# Autodesk Inventor assembly: Carriage Streamlined
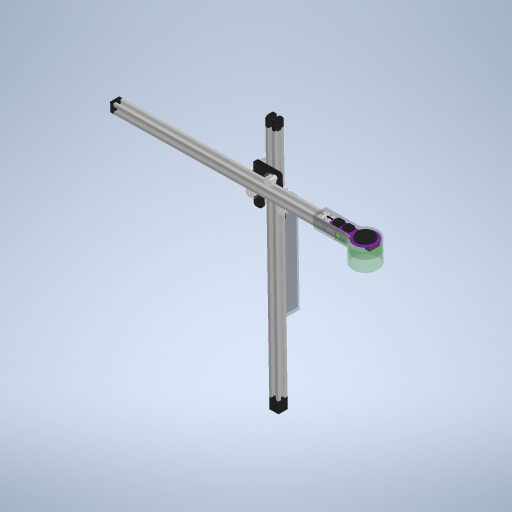
[picture p0: Inventor's stored thumbnail of the model, 512x512]
Saved by Autodesk Inventor 2024 (Build 280153000, 153)
## iProperties
Created: 2022-12-12
Part Number: Carriage Streamlined
Document SubType Name: Assembly
Designer: AdminForWorker
Title: Carriage Streamlined v19
Author: AdminForWorker
## Documents named in this file (23)
- C:\Users\lunima\Desktop\DOSYN\3D Model\Dosyn.iam
- C:\Users\lunima\Desktop\DOSYN\3D Model\Carriage\Routed Spacer.ipt
- C:\Users\lunima\Desktop\DOSYN\3D Model\Carriage\Wheel.iam
- C:\Users\lunima\Desktop\DOSYN\3D Model\Carriage\Wheel_1.iam
- C:\Users\lunima\Desktop\DOSYN\3D Model\Carriage\Wheel_2.iam
- C:\Users\lunima\Desktop\DOSYN\3D Model\Carriage\Wheel_3.iam
- C:\Users\lunima\Desktop\DOSYN\3D Model\Carriage\Wheel_4.iam
- C:\Users\lunima\Desktop\DOSYN\3D Model\Carriage\Wheel_5.iam
- C:\Users\lunima\Desktop\DOSYN\3D Model\Carriage\Carriage.ipt
- C:\Users\lunima\Desktop\DOSYN\3D Model\Carriage\Component8.ipt
- C:\Users\lunima\Desktop\DOSYN\3D Model\Carriage\Belt Clip.ipt
- C:\Users\lunima\Desktop\DOSYN\3D Model\Carriage\Pogo Pin Clip.ipt
- C:\Users\lunima\Desktop\DOSYN\3D Model\Main Structure\2020Z.ipt
- C:\Users\lunima\Desktop\DOSYN\3D Model\Main Structure\Side Lid.ipt
- C:\Users\lunima\Desktop\DOSYN\3D Model\Main Structure\Base.ipt
- C:\Users\lunima\Desktop\DOSYN\3D Model\Main Structure\Pulley Mount.ipt
- C:\Users\lunima\Desktop\DOSYN\3D Model\Counterweight\Counterweight Belt Clip.ipt
- C:\Users\lunima\Desktop\DOSYN\3D Model\Counterweight\Counterweight Enclosure.ipt
- C:\Users\lunima\Desktop\DOSYN\3D Model\Counterweight\Counterweight Flex Tab.ipt
- C:\Users\lunima\Desktop\DOSYN\3D Model\Counterweight\Counterweight Lid.ipt
- C:\Users\lunima\Desktop\DOSYN\3D Model\LED Cover\Dosyn LED.iam
- C:\Users\lunima\Desktop\DOSYN\3D Model\Main Structure\Hot Pipe.ipt
- C:\Users\lunima\Desktop\DOSYN\3D Model\Carriage\Pogo Pin.ipt
## Components (29 placed, 17 different names)
1. Routed Spacer:1 — 旋转:9, 旋转:10
2. Routed Spacer:2 — 旋转:12, 旋转:13
3. Wheel:1 [sub-assembly] — 旋转:13
4. Wheel:2 [sub-assembly] — 旋转:14
5. Wheel:3 [sub-assembly] — 旋转:10
6. Routed Spacer:4 — 旋转:7, 旋转:8
7. Routed Spacer:5 — 旋转:5, 旋转:6
8. Routed Spacer:6 — 刚性:1, 旋转:4
9. Wheel:4 [sub-assembly] — 旋转:8
10. Wheel:5 [sub-assembly] — 旋转:4
11. Wheel:6 [sub-assembly] — 旋转:6
12. Carriage:1 — 旋转:1, 旋转:2, 旋转:3, 刚性:1, 旋转:5, 旋转:7, 旋转:9, 旋转:11, 旋转:12, 配合:1, 配合:2, 表面齐平:1, 配合:3, 表面齐平:2
13. Component8:1 — 旋转:11, 旋转:14
14. Belt Clip:1 — 旋转:1, 配合:1
15. Pogo Pin Clip:1 — 旋转:2
16. Pogo Pin Clip:2 — 旋转:3, 配合:15, 配合:16, 配合:17, 配合:18, 配合:19, 配合:20
17. 2020Z:1 — 配合:3, 表面齐平:2, 旋转:16, 表面齐平:4, 旋转:17, 表面齐平:5, 配合:10, 表面齐平:6
18. 2020Z:2 — 配合:2, 表面齐平:1, 旋转:15, 表面齐平:3, 配合:11, 配合:12, 配合:13, 配合:14, 表面齐平:7
19. Side Lid:1 — 旋转:15, 表面齐平:3
20. Base:1 — 旋转:16, 表面齐平:4
21. Pulley Mount:1 — 旋转:17, 表面齐平:5
22. Counterweight Belt Clip:1 — 旋转:18, 配合:7
23. Counterweight Enclosure:1 — 配合:4, 配合:5, 配合:6, 旋转:18, 配合:7, 配合:8, 配合:9, 配合:10, 表面齐平:6
24. Counterweight Flex Tab:1 — 配合:4, 配合:5, 配合:6
25. Counterweight Lid:1 — 配合:8, 配合:9
26. Dosyn LED:1 [sub-assembly] — 配合:11, 配合:12, 配合:13
27. Hot Pipe:1 — 配合:14, 表面齐平:7
28. Pogo Pin:1 — 配合:15, 配合:16, 配合:17
29. Pogo Pin:2 — 配合:18, 配合:19, 配合:20
## Relationships (46: Mate 20, RevoluteJoint 18, Flush 7, WeldJoint 1)
- 旋转:1 [RevoluteJoint]: Carriage:1 ↔ Belt Clip:1
- 旋转:2 [RevoluteJoint]: Carriage:1 ↔ Pogo Pin Clip:1
- 旋转:3 [RevoluteJoint]: Carriage:1 ↔ Pogo Pin Clip:2
- 刚性:1 [WeldJoint]: Routed Spacer:6 ↔ Carriage:1
- 旋转:4 [RevoluteJoint]: Routed Spacer:6 ↔ Wheel:5
- 旋转:5 [RevoluteJoint]: Routed Spacer:5 ↔ Carriage:1
- 旋转:6 [RevoluteJoint]: Routed Spacer:5 ↔ Wheel:6
- 旋转:7 [RevoluteJoint]: Routed Spacer:4 ↔ Carriage:1
- 旋转:8 [RevoluteJoint]: Routed Spacer:4 ↔ Wheel:4
- 旋转:9 [RevoluteJoint]: Routed Spacer:1 ↔ Carriage:1
- 旋转:10 [RevoluteJoint]: Routed Spacer:1 ↔ Wheel:3
- 旋转:11 [RevoluteJoint]: Carriage:1 ↔ Component8:1
- 旋转:12 [RevoluteJoint]: Routed Spacer:2 ↔ Carriage:1
- 旋转:13 [RevoluteJoint]: Routed Spacer:2 ↔ Wheel:1
- 旋转:14 [RevoluteJoint]: Wheel:2 ↔ Component8:1
- 配合:1 [Mate]: Carriage:1 ↔ Belt Clip:1
- 配合:2 [Mate] (1.5 mm): Carriage:1 ↔ 2020Z:2
- 表面齐平:1 [Flush] (18.85 mm): Carriage:1 ↔ 2020Z:2
- 配合:3 [Mate] (1.5 mm): Carriage:1 ↔ 2020Z:1
- 表面齐平:2 [Flush] (18.85 mm): Carriage:1 ↔ 2020Z:1
- 旋转:15 [RevoluteJoint]: 2020Z:2 ↔ Side Lid:1
- 表面齐平:3 [Flush]: 2020Z:2 ↔ Side Lid:1
- 旋转:16 [RevoluteJoint]: 2020Z:1 ↔ Base:1
- 表面齐平:4 [Flush]: 2020Z:1 ↔ Base:1
- 旋转:17 [RevoluteJoint]: 2020Z:1 ↔ Pulley Mount:1
- 表面齐平:5 [Flush]: 2020Z:1 ↔ Pulley Mount:1
- 配合:4 [Mate]: Counterweight Enclosure:1 ↔ Counterweight Flex Tab:1
- 配合:5 [Mate]: Counterweight Enclosure:1 ↔ Counterweight Flex Tab:1
- 配合:6 [Mate] (0.1 mm): Counterweight Enclosure:1 ↔ Counterweight Flex Tab:1
- 旋转:18 [RevoluteJoint]: Counterweight Belt Clip:1 ↔ Counterweight Enclosure:1
- 配合:7 [Mate]: Counterweight Belt Clip:1 ↔ Counterweight Enclosure:1
- 配合:8 [Mate]: Counterweight Enclosure:1 ↔ Counterweight Lid:1
- 配合:9 [Mate]: Counterweight Enclosure:1 ↔ Counterweight Lid:1
- 配合:10 [Mate]: 2020Z:1 ↔ Counterweight Enclosure:1
- 表面齐平:6 [Flush]: 2020Z:1 ↔ Counterweight Enclosure:1
- 配合:11 [Mate]: 2020Z:2 ↔ Dosyn LED:1
- 配合:12 [Mate] (0.25 mm): 2020Z:2 ↔ Dosyn LED:1
- 配合:13 [Mate]: 2020Z:2 ↔ Dosyn LED:1
- 配合:14 [Mate]: 2020Z:2 ↔ Hot Pipe:1
- 表面齐平:7 [Flush] (-45 mm): 2020Z:2 ↔ Hot Pipe:1
- 配合:15 [Mate]: Pogo Pin Clip:2 ↔ Pogo Pin:1
- 配合:16 [Mate]: Pogo Pin Clip:2 ↔ Pogo Pin:1
- 配合:17 [Mate]: Pogo Pin Clip:2 ↔ Pogo Pin:1
- 配合:18 [Mate]: Pogo Pin Clip:2 ↔ Pogo Pin:2
- 配合:19 [Mate]: Pogo Pin Clip:2 ↔ Pogo Pin:2
- 配合:20 [Mate]: Pogo Pin Clip:2 ↔ Pogo Pin:2
